# Autodesk Inventor assembly: Platine_ZSB
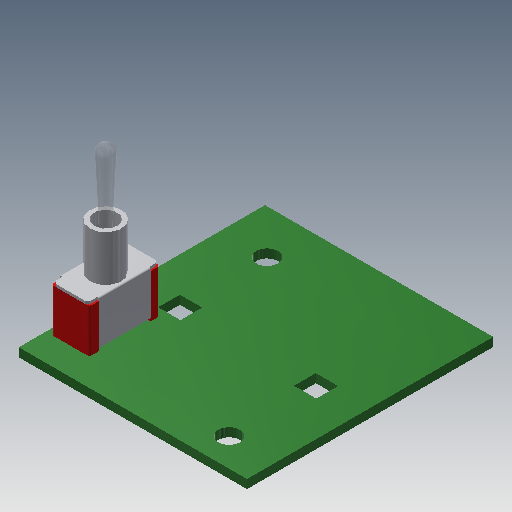
[picture p0: Inventor's stored thumbnail of the model, 512x512]
Saved by Autodesk Inventor 2019 (Build 230136000, 136)
## iProperties
Created: 2022-11-01
Part Number: Platine_ZSB
Material: Generisch
Document SubType Name: Assembly
Designer: RP
Author: RP
## Documents named in this file (3)
- C:\Users\RP\Documents\Inventor\___Projekt_Useless_Box\_Useless_Box\Platine_ZSB.iam
- C:\Users\RP\Documents\Inventor\___Projekt_Useless_Box\_Useless_Box\Schalter.iam
- C:\Users\RP\Documents\Inventor\___Projekt_Useless_Box\_Useless_Box\Platine.ipt
## Components (2 placed, 2 different names)
1. Platine:1 — Fluchtend:3, Fluchtend:4, Fluchtend:5
2. Schalter:1 [sub-assembly]
## Relationships (6: Flush 5, Mate 1)
- [Mate]: Platine:1 ↔ Schalter:1
- [Flush] (1 mm): Platine:1 ↔ Schalter:1
- [Flush] (-5 mm): Platine:1 ↔ Schalter:1
- Fluchtend:3 [Flush]: Platine:1
- Fluchtend:4 [Flush]: Platine:1
- Fluchtend:5 [Flush]: Platine:1
